# Autodesk Inventor assembly: ConveyorFullAssembly
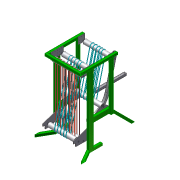
[picture p0: Inventor's stored thumbnail of the model, 180x180]
Saved by Autodesk Inventor 2012 (Build 160160000, 160)
## iProperties
Created: 2012-01-09
Part Number: ConveyorFullAssembly
Document SubType Name: Assembly
Designer: JesseK
Mass: 7637.51 g
Surface Area: 22367.5 cm^2
Volume: 3544 cm^3
Density: 2.15506 g/cm^3
Author: JesseK
## Documents named in this file (9)
- Z:\UserData\Documents\Inventor\team1885frc\Robot2012\Conveyor\ConveyorFullAssembly.iam
- Z:\UserData\Documents\Inventor\team1885frc\Robot2012\Conveyor\ConveyorFrame.iam
- Z:\UserData\Documents\Inventor\team1885frc\Hardware\Bolts\Bolt_0.375_24_1.5len_ButtonHead.ipt
- Z:\UserData\Documents\Inventor\team1885frc\Hardware\Nuts\LockNut_0.375_24.ipt
- Z:\UserData\Documents\Inventor\team1885frc\Robot2012\Conveyor\RollerAssembly.iam
- Z:\UserData\Documents\Inventor\team1885frc\Robot2012\Conveyor\Belt_RearStage2.ipt
- Z:\UserData\Documents\Inventor\team1885frc\Robot2012\Conveyor\Belt_FrontStage2.ipt
- Z:\UserData\Documents\Inventor\team1885frc\Robot2012\Conveyor\Belt_Stage1.ipt
- Z:\UserData\Documents\Inventor\team1885frc\Robot2012\Conveyor\Frame_RearBallGuide.ipt
## Components (50 placed, 8 different names)
1. ConveyorFrame:1 [sub-assembly] — Mate:1, Mate:2, Mate:3, Mate:4, Mate:5, Mate:6, Mate:7, Mate:8, Mate:13, Mate:14, Mate:15, Mate:16, Mate:19, Mate:20, Mate:21, Mate:22, Mate:23, Mate:24, Mate:25, Mate:26, Mate:27, Mate:28, Mate:29, Mate:30, Mate:31, Mate:32, Mate:33, Mate:34, Mate:42, Mate:43, Mate:44, Mate:45, Mate:46, Mate:47, Mate:48, Mate:50, Flush:1
2. Bolt_0.375_24_1.5len_ButtonHead:1 — Mate:1, Mate:2, Mate:12
3. Bolt_0.375_24_1.5len_ButtonHead:2 — Mate:6, Mate:8, Mate:9
4. Bolt_0.375_24_1.5len_ButtonHead:3 — Mate:5, Mate:7, Mate:10
5. Bolt_0.375_24_1.5len_ButtonHead:4 — Mate:3, Mate:4, Mate:11
6. LockNut_0.375_24:1 — Mate:12, Mate:13
7. LockNut_0.375_24:2 — Mate:11, Mate:14
8. LockNut_0.375_24:3 — Mate:10, Mate:16, Mate:18
9. LockNut_0.375_24:4 — Mate:9, Mate:15, Mate:17
10. RollerAssembly:1 [sub-assembly] — Mate:17, Tangent:6, Tangent:7, Tangent:8, Tangent:9, Tangent:10
11. RollerAssembly:2 [sub-assembly] — Mate:18, Tangent:11, Tangent:12, Tangent:13, Tangent:14, Tangent:15, Tangent:16, Tangent:17, Tangent:18
12. RollerAssembly:3 [sub-assembly] — Mate:52, Mate:60, Mate:61, Mate:62, Mate:63, Mate:64
13. RollerAssembly:4 [sub-assembly] — Mate:53, Mate:65, Mate:66, Mate:67, Mate:68, Mate:69, Mate:70, Mate:71, Mate:72
14. RollerAssembly:5 [sub-assembly] — Mate:51, Mate:55, Mate:56, Mate:57, Mate:58, Mate:59
15. RollerAssembly:6 [sub-assembly] — Mate:54, Tangent:1, Tangent:2, Tangent:3, Tangent:4, Tangent:5, Mate:73
16. Bolt_0.375_24_1.5len_ButtonHead:5 — Mate:23, Mate:34, Mate:49
17. Bolt_0.375_24_1.5len_ButtonHead:6 — Mate:26, Mate:27, Mate:39
18. Bolt_0.375_24_1.5len_ButtonHead:7 — Mate:22, Mate:30, Mate:38
19. Bolt_0.375_24_1.5len_ButtonHead:8 — Mate:21, Mate:33, Mate:37
20. Bolt_0.375_24_1.5len_ButtonHead:9 — Mate:20, Mate:32, Mate:36
21. Bolt_0.375_24_1.5len_ButtonHead:10 — Mate:19, Mate:31, Mate:35
22. Bolt_0.375_24_1.5len_ButtonHead:11 — Mate:25, Mate:29, Mate:40
23. Bolt_0.375_24_1.5len_ButtonHead:12 — Mate:24, Mate:28, Mate:41
24. LockNut_0.375_24:5 — Mate:35, Mate:47, Mate:53
25. LockNut_0.375_24:6 — Mate:37, Mate:46, Mate:51
26. LockNut_0.375_24:7 — Mate:36, Mate:45, Mate:52
27. LockNut_0.375_24:8 — Mate:49, Mate:50, Mate:54
28. LockNut_0.375_24:10 — Mate:38, Mate:44
29. LockNut_0.375_24:11 — Mate:41, Mate:42
30. LockNut_0.375_24:12 — Mate:40, Mate:43
31. LockNut_0.375_24:13 — Mate:39, Mate:48
32. Belt_RearStage2:1 — Mate:55, Tangent:1
33. Belt_RearStage2:2 — Mate:56, Tangent:2
34. Belt_RearStage2:3 — Mate:58, Tangent:5
35. Belt_RearStage2:4 — Mate:57, Tangent:3, Flush:2
36. Belt_RearStage2:5 — Mate:59, Tangent:4
37. Belt_FrontStage2:1 — Mate:60, Tangent:6
38. Belt_FrontStage2:2 — Mate:61, Tangent:9
39. Belt_FrontStage2:3 — Mate:62, Tangent:10
40. Belt_FrontStage2:4 — Mate:63, Tangent:7
41. Belt_FrontStage2:5 — Mate:64, Tangent:8
42. Belt_Stage1:2 — Mate:65, Tangent:16
43. Belt_Stage1:3 — Mate:66, Tangent:15
44. Belt_Stage1:4 — Mate:67, Tangent:18
45. Belt_Stage1:5 — Mate:68, Tangent:17
46. Belt_Stage1:6 — Mate:69, Tangent:14
47. Belt_Stage1:7 — Mate:70, Tangent:13
48. Belt_Stage1:8 — Mate:71, Tangent:11
49. Belt_Stage1:9 — Mate:72, Tangent:12
50. Frame_RearBallGuide:1 — Flush:1, Flush:2, Mate:73
## Relationships (93: Mate 73, Tangent 18, Flush 2)
- Mate:1: ConveyorFrame:1 ↔ Bolt_0.375_24_1.5len_ButtonHead:1
- Mate:2: ConveyorFrame:1 ↔ Bolt_0.375_24_1.5len_ButtonHead:1
- Mate:3: ConveyorFrame:1 ↔ Bolt_0.375_24_1.5len_ButtonHead:4
- Mate:4: ConveyorFrame:1 ↔ Bolt_0.375_24_1.5len_ButtonHead:4
- Mate:5: ConveyorFrame:1 ↔ Bolt_0.375_24_1.5len_ButtonHead:3
- Mate:6: ConveyorFrame:1 ↔ Bolt_0.375_24_1.5len_ButtonHead:2
- Mate:7: ConveyorFrame:1 ↔ Bolt_0.375_24_1.5len_ButtonHead:3
- Mate:8: ConveyorFrame:1 ↔ Bolt_0.375_24_1.5len_ButtonHead:2
- Mate:9: Bolt_0.375_24_1.5len_ButtonHead:2 ↔ LockNut_0.375_24:4
- Mate:10: Bolt_0.375_24_1.5len_ButtonHead:3 ↔ LockNut_0.375_24:3
- Mate:11: Bolt_0.375_24_1.5len_ButtonHead:4 ↔ LockNut_0.375_24:2
- Mate:12: Bolt_0.375_24_1.5len_ButtonHead:1 ↔ LockNut_0.375_24:1
- Mate:13: ConveyorFrame:1 ↔ LockNut_0.375_24:1
- Mate:14: ConveyorFrame:1 ↔ LockNut_0.375_24:2
- Mate:15: ConveyorFrame:1 ↔ LockNut_0.375_24:4
- Mate:16: ConveyorFrame:1 ↔ LockNut_0.375_24:3
- Mate:17: LockNut_0.375_24:4 ↔ RollerAssembly:1
- Mate:18: LockNut_0.375_24:3 ↔ RollerAssembly:2
- Mate:19: ConveyorFrame:1 ↔ Bolt_0.375_24_1.5len_ButtonHead:10
- Mate:20: ConveyorFrame:1 ↔ Bolt_0.375_24_1.5len_ButtonHead:9
- Mate:21: ConveyorFrame:1 ↔ Bolt_0.375_24_1.5len_ButtonHead:8
- Mate:22: ConveyorFrame:1 ↔ Bolt_0.375_24_1.5len_ButtonHead:7
- Mate:23: ConveyorFrame:1 ↔ Bolt_0.375_24_1.5len_ButtonHead:5
- Mate:24: ConveyorFrame:1 ↔ Bolt_0.375_24_1.5len_ButtonHead:12
- Mate:25: ConveyorFrame:1 ↔ Bolt_0.375_24_1.5len_ButtonHead:11
- Mate:26: ConveyorFrame:1 ↔ Bolt_0.375_24_1.5len_ButtonHead:6
- Mate:27: ConveyorFrame:1 ↔ Bolt_0.375_24_1.5len_ButtonHead:6
- Mate:28: ConveyorFrame:1 ↔ Bolt_0.375_24_1.5len_ButtonHead:12
- Mate:29: ConveyorFrame:1 ↔ Bolt_0.375_24_1.5len_ButtonHead:11
- Mate:30: ConveyorFrame:1 ↔ Bolt_0.375_24_1.5len_ButtonHead:7
- Mate:31: ConveyorFrame:1 ↔ Bolt_0.375_24_1.5len_ButtonHead:10
- Mate:32: ConveyorFrame:1 ↔ Bolt_0.375_24_1.5len_ButtonHead:9
- Mate:33: ConveyorFrame:1 ↔ Bolt_0.375_24_1.5len_ButtonHead:8
- Mate:34: ConveyorFrame:1 ↔ Bolt_0.375_24_1.5len_ButtonHead:5
- Mate:35: Bolt_0.375_24_1.5len_ButtonHead:10 ↔ LockNut_0.375_24:5
- Mate:36: Bolt_0.375_24_1.5len_ButtonHead:9 ↔ LockNut_0.375_24:7
- Mate:37: Bolt_0.375_24_1.5len_ButtonHead:8 ↔ LockNut_0.375_24:6
- Mate:38: Bolt_0.375_24_1.5len_ButtonHead:7 ↔ LockNut_0.375_24:10
- Mate:39: Bolt_0.375_24_1.5len_ButtonHead:6 ↔ LockNut_0.375_24:13
- Mate:40: Bolt_0.375_24_1.5len_ButtonHead:11 ↔ LockNut_0.375_24:12
- Mate:41: Bolt_0.375_24_1.5len_ButtonHead:12 ↔ LockNut_0.375_24:11
- Mate:42: ConveyorFrame:1 ↔ LockNut_0.375_24:11
- Mate:43: ConveyorFrame:1 ↔ LockNut_0.375_24:12
- Mate:44: ConveyorFrame:1 ↔ LockNut_0.375_24:10
- Mate:45: ConveyorFrame:1 ↔ LockNut_0.375_24:7
- Mate:46: ConveyorFrame:1 ↔ LockNut_0.375_24:6
- Mate:47: ConveyorFrame:1 ↔ LockNut_0.375_24:5
- Mate:48: ConveyorFrame:1 ↔ LockNut_0.375_24:13
- Mate:49: Bolt_0.375_24_1.5len_ButtonHead:5 ↔ LockNut_0.375_24:8
- Mate:50: ConveyorFrame:1 ↔ LockNut_0.375_24:8
- Mate:51: RollerAssembly:5 ↔ LockNut_0.375_24:6
- Mate:52: RollerAssembly:3 ↔ LockNut_0.375_24:7
- Mate:53: RollerAssembly:4 ↔ LockNut_0.375_24:5
- Mate:54: RollerAssembly:6 ↔ LockNut_0.375_24:8
- Mate:55: RollerAssembly:5 ↔ Belt_RearStage2:1
- Tangent:1: RollerAssembly:6 ↔ Belt_RearStage2:1
- Mate:56: RollerAssembly:5 ↔ Belt_RearStage2:2
- Tangent:2: RollerAssembly:6 ↔ Belt_RearStage2:2
- Mate:57: RollerAssembly:5 ↔ Belt_RearStage2:4
- Mate:58: RollerAssembly:5 ↔ Belt_RearStage2:3
- Mate:59: RollerAssembly:5 ↔ Belt_RearStage2:5
- Tangent:3: RollerAssembly:6 ↔ Belt_RearStage2:4
- Tangent:4: RollerAssembly:6 ↔ Belt_RearStage2:5
- Tangent:5: RollerAssembly:6 ↔ Belt_RearStage2:3
- Mate:60: RollerAssembly:3 ↔ Belt_FrontStage2:1
- Tangent:6: RollerAssembly:1 ↔ Belt_FrontStage2:1
- Mate:61: RollerAssembly:3 ↔ Belt_FrontStage2:2
- Mate:62: RollerAssembly:3 ↔ Belt_FrontStage2:3
- Mate:63: RollerAssembly:3 ↔ Belt_FrontStage2:4
- Mate:64: RollerAssembly:3 ↔ Belt_FrontStage2:5
- Tangent:7: RollerAssembly:1 ↔ Belt_FrontStage2:4
- Tangent:8: RollerAssembly:1 ↔ Belt_FrontStage2:5
- Tangent:9: RollerAssembly:1 ↔ Belt_FrontStage2:2
- Tangent:10: RollerAssembly:1 ↔ Belt_FrontStage2:3
- Mate:65: RollerAssembly:4 ↔ Belt_Stage1:2
- Mate:66: RollerAssembly:4 ↔ Belt_Stage1:3
- Mate:67: RollerAssembly:4 ↔ Belt_Stage1:4
- Mate:68: RollerAssembly:4 ↔ Belt_Stage1:5
- Mate:69: RollerAssembly:4 ↔ Belt_Stage1:6
- Mate:70: RollerAssembly:4 ↔ Belt_Stage1:7
- Mate:71: RollerAssembly:4 ↔ Belt_Stage1:8
- Mate:72: RollerAssembly:4 ↔ Belt_Stage1:9
- Tangent:11: RollerAssembly:2 ↔ Belt_Stage1:8
- Tangent:12: RollerAssembly:2 ↔ Belt_Stage1:9
- Tangent:13: RollerAssembly:2 ↔ Belt_Stage1:7
- Tangent:14: RollerAssembly:2 ↔ Belt_Stage1:6
- Tangent:15: RollerAssembly:2 ↔ Belt_Stage1:3
- Tangent:16: RollerAssembly:2 ↔ Belt_Stage1:2
- Tangent:17: RollerAssembly:2 ↔ Belt_Stage1:5
- Tangent:18: RollerAssembly:2 ↔ Belt_Stage1:4
- Flush:1 (-152.4 mm): ConveyorFrame:1 ↔ Frame_RearBallGuide:1
- Flush:2 (190.5 mm): Belt_RearStage2:4 ↔ Frame_RearBallGuide:1
- Mate:73: RollerAssembly:6 ↔ Frame_RearBallGuide:1
